# Autodesk Inventor assembly: Motor
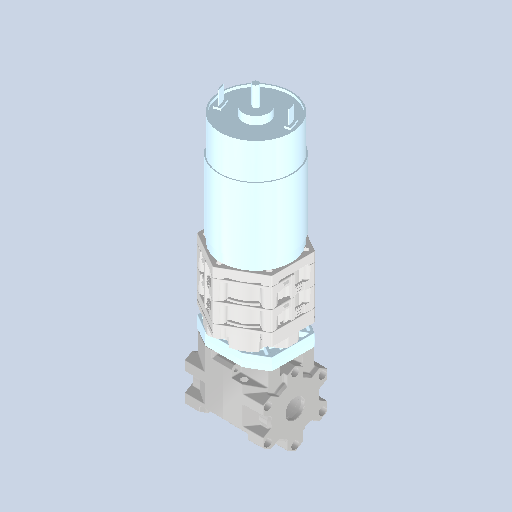
[picture p0: Inventor's stored thumbnail of the model, 512x512]
Saved by Autodesk Inventor 2022.1 (Build 261234020, 234B)
## iProperties
Created: 2022-10-19
Part Number: Motor
Document SubType Name: Assembly
Designer: Alexander
Author: Alexander
## Documents named in this file (8)
- C:\Users\Alexander\Desktop\upload\Octobot\Motor.iam
- C:\Users\Alexander\Desktop\upload\Octobot\Parts\Gearbox1.ipt
- C:\Users\Alexander\Desktop\upload\Octobot\Parts\Gearbox2.ipt
- C:\Users\Alexander\Desktop\upload\Octobot\Parts\Gearbox3.ipt
- C:\Users\Alexander\Desktop\upload\Octobot\Parts\REV-41-1615.ipt
- C:\Users\Alexander\Desktop\upload\Octobot\Parts\REV-41-1607.ipt
- C:\Users\Alexander\Desktop\upload\Octobot\Parts\Motor.ipt
- C:\Users\Alexander\Desktop\upload\Octobot\Parts\REV-41-1601.ipt
## Components (8 placed, 7 different names)
1. REV-41-1601:3 — Mate:8, Mate:9, Mate:10, Mate:11, Mate:12, Mate:13
2. REV-41-1601:4 — Mate:5, Mate:6, Mate:7, Mate:8, Mate:9, Mate:10
3. Gearbox1:1 — Mate:1, Flush:1, Mate:3
4. Gearbox2:1 — Mate:1, Flush:1, Mate:2, Mate:3, Mate:4, Rigid:1
5. Gearbox3:1 — Mate:2, Mate:4
6. REV-41-1615:1 — Rigid:1, Mate:5, Mate:6, Mate:7
7. REV-41-1607:1 — Mate:11, Mate:12, Mate:13, Mate:14, Mate:15
8. Motor:1 — Mate:14, Mate:15
## Relationships (17: Mate 15, Flush 1, WeldJoint 1)
- Mate:1: Gearbox1:1 ↔ Gearbox2:1
- Flush:1: Gearbox1:1 ↔ Gearbox2:1
- Mate:2: Gearbox2:1 ↔ Gearbox3:1
- Mate:3: Gearbox1:1 ↔ Gearbox2:1
- Mate:4: Gearbox2:1 ↔ Gearbox3:1
- Rigid:1 [WeldJoint]: Gearbox2:1 ↔ REV-41-1615:1
- Mate:5: REV-41-1601:4 ↔ REV-41-1615:1
- Mate:6: REV-41-1601:4 ↔ REV-41-1615:1
- Mate:7: REV-41-1601:4 ↔ REV-41-1615:1
- Mate:8: REV-41-1601:3 ↔ REV-41-1601:4
- Mate:9: REV-41-1601:3 ↔ REV-41-1601:4
- Mate:10: REV-41-1601:3 ↔ REV-41-1601:4
- Mate:11: REV-41-1601:3 ↔ REV-41-1607:1
- Mate:12: REV-41-1601:3 ↔ REV-41-1607:1
- Mate:13: REV-41-1601:3 ↔ REV-41-1607:1
- Mate:14: REV-41-1607:1 ↔ Motor:1
- Mate:15: REV-41-1607:1 ↔ Motor:1
